# Autodesk Inventor assembly: Assembly1
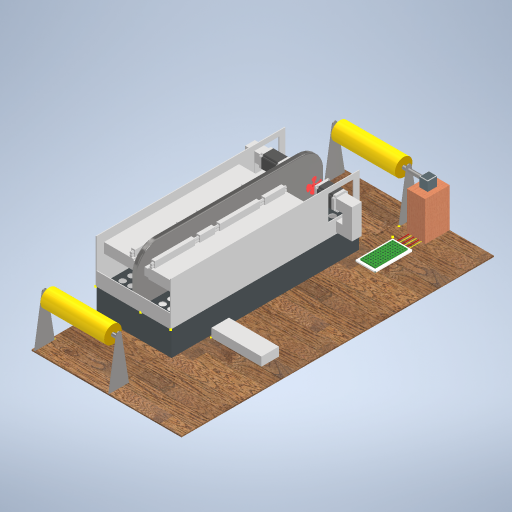
[picture p0: Inventor's stored thumbnail of the model, 512x512]
Saved by Autodesk Inventor 2024 (Build 280153000, 153)
## iProperties
Created: 2024-01-19
Part Number: Assembly1
Document SubType Name: Assembly
Designer: HP
Author: HP
## Documents named in this file (13)
- C:\Users\RAHUL\Desktop\305 cad\Assembly1.iam
- C:\Users\RAHUL\Desktop\305 cad\base.ipt
- C:\Users\RAHUL\Desktop\305 cad\stand.ipt
- C:\Users\RAHUL\Desktop\305 cad\roller.ipt
- C:\Users\RAHUL\Desktop\305 cad\circuit.ipt
- C:\Users\RAHUL\Desktop\305 cad\c_part1.ipt
- C:\Users\RAHUL\Desktop\305 cad\c_part2.ipt
- C:\Users\RAHUL\Desktop\305 cad\stand without motor.ipt
- C:\Users\RAHUL\Desktop\305 cad\Walls_new.ipt
- C:\Users\RAHUL\Desktop\305 cad\fan.ipt
- C:\Users\RAHUL\Desktop\305 cad\motor.ipt
- C:\Users\RAHUL\Desktop\305 cad\motor support.ipt
- C:\Users\RAHUL\Desktop\305 cad\water tank mm.ipt
## Components (16 placed, 12 different names)
1. base:1 — Mate:1, Flush:2, Flush:3, Mate:2, Flush:4, Mate:12, Mate:14, Flush:10, Flush:11, Mate:18, Flush:14, Flush:15, Mate:38
2. stand:1 — Flush:3, Mate:2, Flush:4, Mate:5, Mate:7, Mate:13, Flush:20
3. roller:1 — Mate:17, Mate:19
4. roller:2 — Mate:5, Mate:7
5. circuit:3 — Mate:12, Mate:13, Flush:20
6. c_part1:1 — Mate:14, Flush:10, Flush:11, Mate:15, Flush:12, Flush:13, Mate:21, Mate:22, Flush:16, Mate:37, Flush:19
7. c_part2:1 — Mate:15, Flush:12, Flush:13
8. stand without motor:1 — Mate:17, Mate:18, Mate:19, Flush:14, Flush:15
9. Walls_new:1 — Mate:21, Mate:22, Flush:16, Flush:17, Flush:18, Mate:27, Mate:28, Mate:29, Mate:30
10. fan:1 — Mate:23, Mate:24
11. motor:1 — Mate:23, Mate:24, Flush:17, Mate:29, Mate:30, Mate:31, Mate:32, Mate:33
12. fan:2
13. motor:2 — Flush:18, Mate:27, Mate:28, Mate:34, Mate:35, Mate:36
14. motor support:1 — Mate:31, Mate:32, Mate:33
15. motor support:2 — Mate:34, Mate:35, Mate:36
16. water tank mm:1 — Mate:37, Mate:38, Flush:19
## Relationships (43: Mate 29, Flush 14)
- Mate:1: base:1
- Flush:2 (-500 mm): base:1
- Flush:3: base:1 ↔ stand:1
- Mate:2: base:1 ↔ stand:1
- Flush:4 (10 mm): base:1 ↔ stand:1
- Mate:5: stand:1 ↔ roller:2
- Mate:7 (20 mm): stand:1 ↔ roller:2
- Mate:12: base:1 ↔ circuit:3
- Mate:13 (50 mm): stand:1 ↔ circuit:3
- Mate:14: base:1 ↔ c_part1:1
- Flush:10 (250 mm): base:1 ↔ c_part1:1
- Flush:11 (10 mm): base:1 ↔ c_part1:1
- Mate:15: c_part1:1 ↔ c_part2:1
- Flush:12: c_part1:1 ↔ c_part2:1
- Flush:13 (140 mm): c_part1:1 ↔ c_part2:1
- Mate:17: roller:1 ↔ stand without motor:1
- Mate:18: base:1 ↔ stand without motor:1
- Mate:19 (17.5 mm): roller:1 ↔ stand without motor:1
- Flush:14 (10 mm): base:1 ↔ stand without motor:1
- Flush:15 (35 mm): base:1 ↔ stand without motor:1
- Mate:21: c_part1:1 ↔ Walls_new:1
- Mate:22: c_part1:1 ↔ Walls_new:1
- Flush:16: c_part1:1 ↔ Walls_new:1
- Mate:23: fan:1 ↔ motor:1
- Mate:24: fan:1 ↔ motor:1
- [Mate]: fan:2 ↔ motor:2
- [Mate]: fan:2 ↔ motor:2
- Flush:17: Walls_new:1 ↔ motor:1
- Flush:18: Walls_new:1 ↔ motor:2
- Mate:27 (22 mm): Walls_new:1 ↔ motor:2
- Mate:28 (22 mm): Walls_new:1 ↔ motor:2
- Mate:29 (22 mm): Walls_new:1 ↔ motor:1
- Mate:30 (22 mm): Walls_new:1 ↔ motor:1
- Mate:31: motor:1 ↔ motor support:1
- Mate:32 (8.5 mm): motor:1 ↔ motor support:1
- Mate:33 (8.5 mm): motor:1 ↔ motor support:1
- Mate:34: motor:2 ↔ motor support:2
- Mate:35 (8.5 mm): motor:2 ↔ motor support:2
- Mate:36 (8.5 mm): motor:2 ↔ motor support:2
- Mate:37: c_part1:1 ↔ water tank mm:1
- Mate:38: base:1 ↔ water tank mm:1
- Flush:19 (150 mm): c_part1:1 ↔ water tank mm:1
- Flush:20: stand:1 ↔ circuit:3
## Named parameters: d57_d55 = 0 mm, d58_d56 = 0 mm
